# Autodesk Inventor assembly: Static_foot_V02
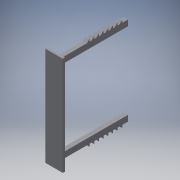
[picture p0: Inventor's stored thumbnail of the model, 180x180]
Saved by Autodesk Inventor 2019.4 (Build 234330000, 330)
## iProperties
Created: 2019-12-18
Part Number: Static_foot_V02
Document SubType Name: Assembly
Designer: fabfarm
Author: fabfarm
## Documents named in this file (3)
- D:\Users\fabfarm\Documents\Saw table\Static_foot_V02.iam
- D:\Users\fabfarm\Documents\Saw table\floor_Part.ipt
- D:\Users\fabfarm\Documents\Saw table\graduated_foot_02.ipt
## Components (5 placed, 2 different names)
1. floor_Part:1 — Mate:2, Mate:3, Mate:4, Mate:6, Mate:7, Mate:8
2. graduated_foot_02:1 — Mate:5, Flush:3, Flush:4, Mate:8
3. graduated_foot_02:2 — Mate:5, Flush:3, Flush:4, Mate:6, Mate:7
4. graduated_foot_02:3 — Mate:1, Flush:1, Flush:2, Mate:2, Mate:4
5. graduated_foot_02:4 — Mate:1, Flush:1, Flush:2, Mate:3
## Relationships (12: Mate 8, Flush 4)
- Mate:1: graduated_foot_02:3 ↔ graduated_foot_02:4
- Flush:1: graduated_foot_02:3 ↔ graduated_foot_02:4
- Flush:2: graduated_foot_02:3 ↔ graduated_foot_02:4
- Mate:2: floor_Part:1 ↔ graduated_foot_02:3
- Mate:3: floor_Part:1 ↔ graduated_foot_02:4
- Mate:4: floor_Part:1 ↔ graduated_foot_02:3
- Mate:5: graduated_foot_02:1 ↔ graduated_foot_02:2
- Flush:3: graduated_foot_02:1 ↔ graduated_foot_02:2
- Flush:4: graduated_foot_02:1 ↔ graduated_foot_02:2
- Mate:6: floor_Part:1 ↔ graduated_foot_02:2
- Mate:7: floor_Part:1 ↔ graduated_foot_02:2
- Mate:8: floor_Part:1 ↔ graduated_foot_02:1
